# Autodesk Inventor assembly: Lift
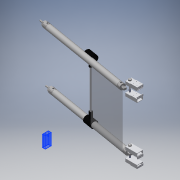
[picture p0: Inventor's stored thumbnail of the model, 180x180]
Saved by Autodesk Inventor 2016 (Build 200138000, 138)
## iProperties
Created: 2016-01-16
Part Number: Lift
Description: STEP AP214
Document SubType Name: Assembly
Designer: Douglas
Sending System: SolidWorks 2015
Preprocessor: SwSTEP 2.0
Title: Lift.STEP
Revision Number: ANY
## Documents named in this file (10)
- D:\SkyDrive\GitHub\2016-Robot-CAD\Inventor\Lift.iam
- D:\Desktop\am-2954 AM14U2 2x3 Hole Bracket.ipt
- D:\Desktop\Piston Holder.ipt
- D:\Desktop\27 in Piston.iam
- D:\Desktop\Pneumatic pivot bar.ipt
- D:\Desktop\10mm Shaft Collar.ipt
- D:\Desktop\Pneumatic Spacer.ipt
- D:\Desktop\Pneumatic Brace Mount.ipt
- D:\Desktop\Pneumatic Brace Bar.ipt
- D:\Desktop\Sponser Lexan Sheet.ipt
## Components (24 placed, 24 different names)
1. am-2954 AM14U2 2x3 Hole Bracket_1
2. am-2954 AM14U2 2x3 Hole Bracket_2
3. Piston Holder_3
4. am-2954 AM14U2 2x3 Hole Bracket_4
5. am-2954 AM14U2 2x3 Hole Bracket_5
6. Piston Holder_6
7. 27 in Piston_7 [sub-assembly]
8. 27 in Piston_8 [sub-assembly]
9. Piston Holder_9 — Mate:1, Mate:2
10. Piston Holder_10
11. Pneumatic pivot bar_11 — Mate:1, Mate:3
12. Pneumatic pivot bar_12
13. 10mm Shaft Collar_13
14. 10mm Shaft Collar_14
15. 10mm Shaft Collar_15 — Mate:2, Mate:3
16. 10mm Shaft Collar_16
17. Pneumatic Spacer_17
18. Pneumatic Spacer_18
19. Pneumatic Spacer_19
20. Pneumatic Spacer_20
21. Pneumatic Brace Mount_21
22. Pneumatic Brace Mount_22
23. Pneumatic Brace Bar_23
24. Sponser Lexan Sheet_24
## Relationships (3: Mate 3)
- Mate:1: Piston Holder_9 ↔ Pneumatic pivot bar_11
- Mate:2: Piston Holder_9 ↔ 10mm Shaft Collar_15
- Mate:3: Pneumatic pivot bar_11 ↔ 10mm Shaft Collar_15
